# Autodesk Inventor assembly: lift frame
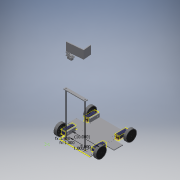
[picture p0: Inventor's stored thumbnail of the model, 180x180]
Saved by Autodesk Inventor 2019 (Build 230136000, 136)
## iProperties
Created: 2018-09-29
Part Number: lift frame
Document SubType Name: Assembly
Designer: User
Author: User
## Documents named in this file (11)
- C:\Robotics\CAD\2018-19_CAD\lift\lift frame.iam
- C:\Robotics\CAD\2017-18_CAD\Prototypes\Gen2PlatePart.ipt
- C:\Robotics\CAD\2017-18_CAD\Prototypes\MotorHolderA.ipt
- C:\Robotics\CAD\2017-18_CAD\Prototypes\MotorHolderB.ipt
- C:\Robotics\CAD\COTSParts\Wheels\am-2648_4inWheel8mmHub.ipt
- C:\Robotics\CAD\COTSParts\Rev\REV-41-1300HexMotor.ipt
- C:\Robotics\CAD\2018-19_CAD\lift\meet 1 lift\Part3.ipt
- C:\Robotics\CAD\2018-19_CAD\lift\lift bar.ipt
- lift bar.ipt
- C:\Robotics\CAD\2018-19_CAD\lift\lift box.ipt
- C:\Robotics\CAD\2018-19_CAD\smart servo with servo block.iam
## Components (18 placed, 9 different names)
1. Gen2PlatePart:1 — Mate:1, Mate:4, Mate:7, Mate:8, Mate:9, Mate:10, Mate:11, Mate:12, Mate:13, Mate:14, Mate:17, Mate:18, Mate:26, Mate:27, Mate:28, Mate:29, Mate:32, Flush:5
2. MotorHolderA:1 — Mate:7, Mate:8, Mate:9, Mate:23, Mate:24, Angle:4
3. MotorHolderA:2 — Mate:4, Mate:13, Mate:14, Mate:15, Mate:16, Angle:1
4. MotorHolderB:1 — Mate:10, Mate:11, Mate:12, Mate:21, Mate:22, Angle:3
5. MotorHolderB:2 — Mate:1, Mate:17, Mate:18, Mate:19, Mate:20, Angle:2
6. am-2648_4inWheel8mmHub:1 — Mate:25
7. REV-41-1300HexMotor:1 — Mate:21, Mate:22, Angle:3, Insert:2
8. REV-41-1300HexMotor:2 — Mate:19, Mate:20, Angle:2, Insert:4
9. REV-41-1300HexMotor:3 — Mate:15, Mate:16, Angle:1, Mate:25
10. REV-41-1300HexMotor:4 — Mate:23, Mate:24, Angle:4, Insert:3
11. am-2648_4inWheel8mmHub:2 — Insert:4
12. am-2648_4inWheel8mmHub:3 — Insert:3
13. am-2648_4inWheel8mmHub:4 — Insert:2
14. Part3:1 — Mate:26, Mate:28, Mate:31, Mate:33
15. Part3:2 — Mate:27, Mate:29, Mate:30
16. lift bar:1 — Mate:30, Mate:31, Mate:32, Flush:4
17. lift box:1 — Insert:5, Flush:4, Mate:33
18. smart servo with servo block:1 [sub-assembly] — Insert:5, Flush:5
## Relationships (39: Mate 29, Angle 4, Insert 4, Flush 2)
- Mate:1: Gen2PlatePart:1 ↔ MotorHolderB:2
- Mate:4: Gen2PlatePart:1 ↔ MotorHolderA:2
- Mate:7: Gen2PlatePart:1 ↔ MotorHolderA:1
- Mate:8: Gen2PlatePart:1 ↔ MotorHolderA:1
- Mate:9: Gen2PlatePart:1 ↔ MotorHolderA:1
- Mate:10: Gen2PlatePart:1 ↔ MotorHolderB:1
- Mate:11: Gen2PlatePart:1 ↔ MotorHolderB:1
- Mate:12: Gen2PlatePart:1 ↔ MotorHolderB:1
- Mate:13: Gen2PlatePart:1 ↔ MotorHolderA:2
- Mate:14: Gen2PlatePart:1 ↔ MotorHolderA:2
- Mate:15: MotorHolderA:2 ↔ REV-41-1300HexMotor:3
- Mate:16: MotorHolderA:2 ↔ REV-41-1300HexMotor:3
- Angle:1 (180 deg): MotorHolderA:2 ↔ REV-41-1300HexMotor:3
- Mate:17: Gen2PlatePart:1 ↔ MotorHolderB:2
- Mate:18: Gen2PlatePart:1 ↔ MotorHolderB:2
- Mate:19: MotorHolderB:2 ↔ REV-41-1300HexMotor:2
- Mate:20: MotorHolderB:2 ↔ REV-41-1300HexMotor:2
- Angle:2 (180 deg): MotorHolderB:2 ↔ REV-41-1300HexMotor:2
- Mate:21: MotorHolderB:1 ↔ REV-41-1300HexMotor:1
- Mate:22: MotorHolderB:1 ↔ REV-41-1300HexMotor:1
- Angle:3 (180 deg): MotorHolderB:1 ↔ REV-41-1300HexMotor:1
- Mate:23: MotorHolderA:1 ↔ REV-41-1300HexMotor:4
- Mate:24: MotorHolderA:1 ↔ REV-41-1300HexMotor:4
- Angle:4 (180 deg): MotorHolderA:1 ↔ REV-41-1300HexMotor:4
- Insert:2 (11.43 mm): REV-41-1300HexMotor:1 ↔ am-2648_4inWheel8mmHub:4
- Mate:25 (11.43 mm): am-2648_4inWheel8mmHub:1 ↔ REV-41-1300HexMotor:3
- Insert:3 (11.43 mm): REV-41-1300HexMotor:4 ↔ am-2648_4inWheel8mmHub:3
- Insert:4 (11.43 mm): REV-41-1300HexMotor:2 ↔ am-2648_4inWheel8mmHub:2
- Mate:26: Gen2PlatePart:1 ↔ Part3:1
- Mate:27: Gen2PlatePart:1 ↔ Part3:2
- Mate:28: Gen2PlatePart:1 ↔ Part3:1
- Mate:29: Gen2PlatePart:1 ↔ Part3:2
- Mate:30: Part3:2 ↔ lift bar:1
- Mate:31: Part3:1 ↔ lift bar:1
- Mate:32: Gen2PlatePart:1 ↔ lift bar:1
- Insert:5: lift box:1 ↔ smart servo with servo block:1
- Flush:4 (-400.05 mm): lift bar:1 ↔ lift box:1
- Flush:5 (6.35 mm): Gen2PlatePart:1 ↔ smart servo with servo block:1
- Mate:33 (31.75 mm): Part3:1 ↔ lift box:1
